# Autodesk Inventor assembly: Well's Idea
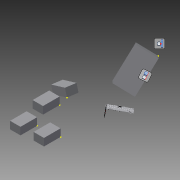
[picture p0: Inventor's stored thumbnail of the model, 180x180]
Saved by Autodesk Inventor 2015 (Build 190159000, 159)
## iProperties
Created: 2015-01-09
Part Number: Well's Idea
Document SubType Name: Assembly
Designer: harrykuperstein
Author: harrykuperstein
## Documents named in this file (5)
- C:\team3556-cad-2015\Well's Idea.iam
- C:\team3556-cad-2015\KOP 2015 CAD\Drive Base CAD\DB_DriveBaseLong_AM14U2.iam.iam
- C:\team3556-cad-2015\Crate.ipt
- C:\team3556-cad-2015\Crate Stacker.ipt
- DB_DriveBaseLong_AM14U2.iam
## Components (6 placed, 3 different names)
1. DB_DriveBaseLong_AM14U2.iam:1 [sub-assembly] — Angle:1, Flush:1, Tangent:1
2. Crate:1
3. Crate:2
4. Crate:3
5. Crate:4
6. Crate Stacker:1 — Angle:1, Flush:1, Tangent:1
## Relationships (3: Angle 1, Flush 1, Tangent 1)
- Angle:1 (68 deg): DB_DriveBaseLong_AM14U2.iam:1 ↔ Crate Stacker:1
- Flush:1: DB_DriveBaseLong_AM14U2.iam:1 ↔ Crate Stacker:1
- Tangent:1 (1981.2 mm): DB_DriveBaseLong_AM14U2.iam:1 ↔ Crate Stacker:1
